# Autodesk Inventor assembly: Femto
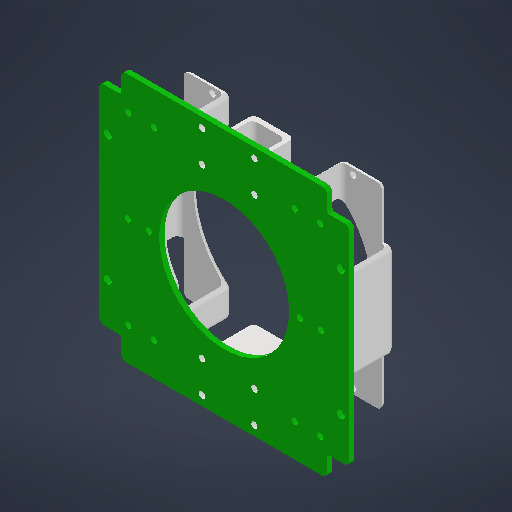
[picture p0: Inventor's stored thumbnail of the model, 512x512]
Saved by Autodesk Inventor 2026.1 (Build 301233020, 233B)
## iProperties
Created: 2025-11-06
Part Number: Femto
Document SubType Name: Assembly
Designer: SPEL
Author: SPEL
## Documents named in this file (4)
- C:\Users\patri\Desktop\SPEL\Femto\CAD\Femto.iam
- C:\Users\patri\Desktop\SPEL\Femto\CAD\PCB.ipt
- C:\Users\patri\Desktop\SPEL\Femto\CAD\soporte inyector completo.ipt
- C:\Users\patri\Desktop\SPEL\Femto\CAD\soporte cerradura.ipt
## Components (5 placed, 3 different names)
1. PCB:1 — Insertar:3, Insertar:4, Insertar:5, Insertar:6, Insertar:7, Insertar:8, Insertar:9, Insertar:10
2. soporte inyector completo:1 — Insertar:3, Insertar:4
3. soporte inyector completo:2 — Insertar:5, Insertar:6
4. soporte cerradura:1 — Insertar:9, Insertar:10
5. soporte cerradura:2 — Insertar:7, Insertar:8
## Relationships (8: Insert 8)
- Insertar:3: PCB:1 ↔ soporte inyector completo:1
- Insertar:4: PCB:1 ↔ soporte inyector completo:1
- Insertar:5: PCB:1 ↔ soporte inyector completo:2
- Insertar:6: PCB:1 ↔ soporte inyector completo:2
- Insertar:7: PCB:1 ↔ soporte cerradura:2
- Insertar:8: PCB:1 ↔ soporte cerradura:2
- Insertar:9: PCB:1 ↔ soporte cerradura:1
- Insertar:10: PCB:1 ↔ soporte cerradura:1
